# Autodesk Inventor assembly: Lift assembly left
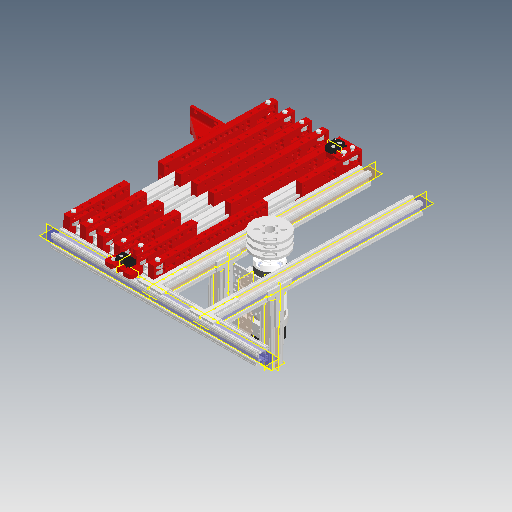
[picture p0: Inventor's stored thumbnail of the model, 512x512]
Saved by Autodesk Inventor 2020 (Build 240168000, 168)
## iProperties
Created: 2019-11-17
Part Number: Lift assembly left
Document SubType Name: Assembly
Designer: ball
Author: ball
## Documents named in this file (22)
- C:\FTC\FTC8863CAD\2019 Robot\Delivery\Lift assembly left.iam
- C:\FTC\FTC8863CAD\Actobotics\605 parts\605630.ipt
- C:\FTC\FTC8863CAD\StepLibraries\Nuts\2-56 NYLON-INSERT LOCKNUT.ipt
- C:\FTC\FTC8863CAD\StepLibraries\Screws\M3 x 25 HEX HEAD CAP SCREW.ipt
- C:\FTC\FTC8863CAD\2019 Robot\Delivery\Limit switch trigger spacer.ipt
- C:\FTC\FTC8863CAD\Actobotics\565 parts\565046.ipt
- C:\FTC\FTC8863CAD\Actobotics\585 parts\585075.ipt
- C:\FTC\FTC8863CAD\Actobotics\565 parts\xrail_3.5in.ipt
- C:\FTC\FTC8863CAD\Andymark\am-3461a NeveRest 4 with Motor REV3.ipt
- C:\FTC\FTC8863CAD\Actobotics\555 parts\555116 assembly.ipt
- C:\FTC\FTC8863CAD\2019 Robot\Generic Parts\limit switch mount to xrail.ipt
- C:\FTC\FTC8863CAD\StepLibraries\Screws\2-56x.5_18-8 SS PAN HEAD PHILLIPS MACHINE SCREW.ipt
- C:\FTC\FTC8863CAD\StepLibraries\Screws\6-32x.375_18-8 SS TRUSS HEAD PHILLIPS MACHINE SCREW.ipt
- C:\FTC\FTC8863CAD\2019 Robot\Delivery\Limit switch top + mount.iam
- C:\FTC\FTC8863CAD\2019 Robot\Delivery\Coupler lift long left bracket + pulleys.iam
- C:\FTC\FTC8863CAD\2019 Robot\Delivery\SAR330  x 5 + couplers left.iam
- C:\FTC\FTC8863CAD\2019 Robot\Delivery\Coupler lift short left + pulleys.iam
- C:\FTC\FTC8863CAD\Actobotics\615 parts\615468 inner plate.ipt
- C:\FTC\FTC8863CAD\Actobotics\615 parts\615468 outer plate 2_0 diameter.ipt
- C:\FTC\FTC8863CAD\Actobotics\545 parts\545619 assembly.ipt
- C:\FTC\FTC8863CAD\Actobotics\585 parts\585721.ipt
- C:\FTC\FTC8863CAD\2019 Robot\Delivery\Cross bar bracket.ipt
## Components (36 placed, 21 different names)
1. SAR330  x 5 + couplers left:1 [sub-assembly] — Mate:5, Flush:7, Mate:18, Mate:19, Mate:33, Mate:34, Mate:35, Mate:36, Flush:16, Mate:38, Flush:20, Mate:40, Flush:21, Flush:24, Mate:43, Flush:34, Flush:35, Mate:68, Mate:72, Mate:73, Mate:74
2. 605630:2 — Mate:5, Flush:7, Flush:33, Mate:61, Mate:63, Mate:64, Mate:65
3. M3 x 25 HEX HEAD CAP SCREW:1 — Mate:18, Mate:19, Mate:25, Mate:26
4. Limit switch trigger spacer:1 — Mate:25, Mate:26
5. M3 x 25 HEX HEAD CAP SCREW:2 — Mate:33
6. M3 x 25 HEX HEAD CAP SCREW:3 — Mate:34
7. Coupler lift short left + pulleys:1 [sub-assembly] — Mate:35, Mate:36, Flush:16, Flush:17, Flush:19, Mate:37
8. 565046:1 — Flush:17, Flush:19, Mate:37, Mate:39, Flush:22, Mate:42, Flush:25, Mate:48, Mate:49, Mate:60, Flush:32
9. 585075:1 — Mate:38, Flush:20, Mate:39
10. xrail_3.5in:1 — Mate:40, Flush:21, Flush:22, Mate:41, Flush:23, Flush:27, Symmetry:1, Flush:29
11. 585075:2 — Mate:41, Flush:23, Flush:24
12. 565046:2 — Mate:42, Flush:25, Mate:43, Mate:44, Flush:26, Mate:46, Flush:28, Mate:50, Mate:51, Mate:99
13. xrail_3.5in:2 — Mate:44, Flush:26, Flush:27, Mate:45, Mate:47, Mate:52, Symmetry:1, Mate:56, Mate:57, Mate:98, Mate:100, Mate:102
14. 585075:3 — Mate:45, Mate:46, Mate:47
15. 585075:4 — Mate:48, Flush:28, Mate:49
16. 585075:5 — Mate:50, Mate:51, Mate:52
17. am-3461a NeveRest 4 with Motor REV3:1 — Mate:53, Flush:29, Mate:54, Mate:55, Flush:30, Flush:31, Mate:90, Mate:91
18. 555116 assembly:1 — Mate:54, Flush:31
19. 555116 assembly:2 — Mate:55, Flush:30, Mate:56, Mate:57, Mate:103
20. limit switch mount to xrail:1 — Mate:60, Flush:32, Flush:33, Mate:61, Mate:62, Angle:1, Mate:66, Mate:67
21. 2-56 NYLON-INSERT LOCKNUT:4 — Mate:62, Mate:63, Angle:1
22. 2-56x.5_18-8 SS PAN HEAD PHILLIPS MACHINE SCREW:1 — Mate:64, Mate:65
23. 6-32x.375_18-8 SS TRUSS HEAD PHILLIPS MACHINE SCREW:1 — Mate:66, Mate:67
24. Limit switch top + mount:1 [sub-assembly] — Flush:34, Flush:35, Mate:68
25. Coupler lift long left bracket + pulleys:1 [sub-assembly] — Mate:72, Mate:73, Mate:74, Mate:104, Mate:105
26. 615468 inner plate:1 — Mate:76, Mate:77, Mate:78, Mate:79
27. 615468 outer plate 2_0 diameter:1 — Mate:78, Mate:79, Mate:84, Mate:85
28. 615468 inner plate:2 — Mate:76, Mate:77, Mate:80, Mate:81
29. 615468 outer plate 2_0 diameter:2 — Mate:80, Mate:81, Mate:91
30. 615468 inner plate:3 — Mate:82, Mate:83, Mate:84, Mate:86, Mate:87
31. 615468 inner plate:4 — Mate:82, Mate:83, Mate:85
32. 615468 outer plate 2_0 diameter:3 — Mate:86, Mate:87, Mate:88, Mate:89
33. 545619 assembly:1 — Mate:88, Mate:89, Mate:90
34. 585721:1 — Mate:98, Mate:99, Flush:38, Mate:101, Mate:103
35. 585721:2 — Mate:100, Flush:38, Mate:101, Mate:102
36. Cross bar bracke leftt:1 — Mate:104, Mate:105
## Relationships (89: Mate 66, Flush 21, Symmetry 1, Angle 1)
- Mate:5 (1.27 mm): SAR330  x 5 + couplers left:1 ↔ 605630:2
- Flush:7: SAR330  x 5 + couplers left:1 ↔ 605630:2
- Mate:18: SAR330  x 5 + couplers left:1 ↔ M3 x 25 HEX HEAD CAP SCREW:1
- Mate:19 (6 mm): SAR330  x 5 + couplers left:1 ↔ M3 x 25 HEX HEAD CAP SCREW:1
- Mate:25: M3 x 25 HEX HEAD CAP SCREW:1 ↔ Limit switch trigger spacer:1
- Mate:26: M3 x 25 HEX HEAD CAP SCREW:1 ↔ Limit switch trigger spacer:1
- Mate:33: SAR330  x 5 + couplers left:1 ↔ M3 x 25 HEX HEAD CAP SCREW:2
- Mate:34: SAR330  x 5 + couplers left:1 ↔ M3 x 25 HEX HEAD CAP SCREW:3
- Mate:35: SAR330  x 5 + couplers left:1 ↔ Coupler lift short left + pulleys:1
- Mate:36: SAR330  x 5 + couplers left:1 ↔ Coupler lift short left + pulleys:1
- Flush:16: SAR330  x 5 + couplers left:1 ↔ Coupler lift short left + pulleys:1
- Flush:17: Coupler lift short left + pulleys:1 ↔ 565046:1
- Flush:19: Coupler lift short left + pulleys:1 ↔ 565046:1
- Mate:37: Coupler lift short left + pulleys:1 ↔ 565046:1
- Mate:38: SAR330  x 5 + couplers left:1 ↔ 585075:1
- Flush:20: SAR330  x 5 + couplers left:1 ↔ 585075:1
- Mate:39: 565046:1 ↔ 585075:1
- Mate:40: SAR330  x 5 + couplers left:1 ↔ xrail_3.5in:1
- Flush:21: SAR330  x 5 + couplers left:1 ↔ xrail_3.5in:1
- Flush:22 (100.2792 mm): 565046:1 ↔ xrail_3.5in:1
- Mate:41: xrail_3.5in:1 ↔ 585075:2
- Flush:23: xrail_3.5in:1 ↔ 585075:2
- Flush:24: SAR330  x 5 + couplers left:1 ↔ 585075:2
- Mate:42: 565046:1 ↔ 565046:2
- Flush:25: 565046:1 ↔ 565046:2
- Mate:43 (57.15 mm): SAR330  x 5 + couplers left:1 ↔ 565046:2
- Mate:44: 565046:2 ↔ xrail_3.5in:2
- Flush:26: 565046:2 ↔ xrail_3.5in:2
- Flush:27: xrail_3.5in:1 ↔ xrail_3.5in:2
- Mate:45: xrail_3.5in:2 ↔ 585075:3
- Mate:46: 565046:2 ↔ 585075:3
- Mate:47: xrail_3.5in:2 ↔ 585075:3
- Mate:48: 565046:1 ↔ 585075:4
- Flush:28: 565046:2 ↔ 585075:4
- Mate:49: 565046:1 ↔ 585075:4
- Mate:50: 565046:2 ↔ 585075:5
- Mate:51: 565046:2 ↔ 585075:5
- Mate:52: xrail_3.5in:2 ↔ 585075:5
- Symmetry:1: xrail_3.5in:1 ↔ xrail_3.5in:2
- Mate:53: am-3461a NeveRest 4 with Motor REV3:1
- Flush:29: xrail_3.5in:1 ↔ am-3461a NeveRest 4 with Motor REV3:1
- Mate:54: am-3461a NeveRest 4 with Motor REV3:1 ↔ 555116 assembly:1
- Mate:55: am-3461a NeveRest 4 with Motor REV3:1 ↔ 555116 assembly:2
- Flush:30 (19.05 mm): am-3461a NeveRest 4 with Motor REV3:1 ↔ 555116 assembly:2
- Flush:31 (22.86 mm): am-3461a NeveRest 4 with Motor REV3:1 ↔ 555116 assembly:1
- Mate:56: xrail_3.5in:2 ↔ 555116 assembly:2
- Mate:57: xrail_3.5in:2 ↔ 555116 assembly:2
- Mate:60: 565046:1 ↔ limit switch mount to xrail:1
- Flush:32: 565046:1 ↔ limit switch mount to xrail:1
- Flush:33: 605630:2 ↔ limit switch mount to xrail:1
- Mate:61: 605630:2 ↔ limit switch mount to xrail:1
- Mate:62: limit switch mount to xrail:1 ↔ 2-56 NYLON-INSERT LOCKNUT:4
- Mate:63: 605630:2 ↔ 2-56 NYLON-INSERT LOCKNUT:4
- Angle:1 (0 deg): limit switch mount to xrail:1 ↔ 2-56 NYLON-INSERT LOCKNUT:4
- Mate:64: 605630:2 ↔ 2-56x.5_18-8 SS PAN HEAD PHILLIPS MACHINE SCREW:1
- Mate:65: 605630:2 ↔ 2-56x.5_18-8 SS PAN HEAD PHILLIPS MACHINE SCREW:1
- Mate:66: limit switch mount to xrail:1 ↔ 6-32x.375_18-8 SS TRUSS HEAD PHILLIPS MACHINE SCREW:1
- Mate:67: limit switch mount to xrail:1 ↔ 6-32x.375_18-8 SS TRUSS HEAD PHILLIPS MACHINE SCREW:1
- Flush:34: SAR330  x 5 + couplers left:1 ↔ Limit switch top + mount:1
- Flush:35 (2.54 mm): SAR330  x 5 + couplers left:1 ↔ Limit switch top + mount:1
- Mate:68: SAR330  x 5 + couplers left:1 ↔ Limit switch top + mount:1
- Mate:72: SAR330  x 5 + couplers left:1 ↔ Coupler lift long left bracket + pulleys:1
- Mate:73: SAR330  x 5 + couplers left:1 ↔ Coupler lift long left bracket + pulleys:1
- Mate:74: SAR330  x 5 + couplers left:1 ↔ Coupler lift long left bracket + pulleys:1
- Mate:76: 615468 inner plate:1 ↔ 615468 inner plate:2
- Mate:77: 615468 inner plate:1 ↔ 615468 inner plate:2
- Mate:78: 615468 inner plate:1 ↔ 615468 outer plate 2_0 diameter:1
- Mate:79: 615468 inner plate:1 ↔ 615468 outer plate 2_0 diameter:1
- Mate:80: 615468 inner plate:2 ↔ 615468 outer plate 2_0 diameter:2
- Mate:81: 615468 inner plate:2 ↔ 615468 outer plate 2_0 diameter:2
- Mate:82: 615468 inner plate:3 ↔ 615468 inner plate:4
- Mate:83: 615468 inner plate:3 ↔ 615468 inner plate:4
- Mate:84: 615468 outer plate 2_0 diameter:1 ↔ 615468 inner plate:3
- Mate:85: 615468 outer plate 2_0 diameter:1 ↔ 615468 inner plate:4
- Mate:86: 615468 inner plate:3 ↔ 615468 outer plate 2_0 diameter:3
- Mate:87: 615468 inner plate:3 ↔ 615468 outer plate 2_0 diameter:3
- Mate:88: 615468 outer plate 2_0 diameter:3 ↔ 545619 assembly:1
- Mate:89: 615468 outer plate 2_0 diameter:3 ↔ 545619 assembly:1
- Mate:90: am-3461a NeveRest 4 with Motor REV3:1 ↔ 545619 assembly:1
- Mate:91: am-3461a NeveRest 4 with Motor REV3:1 ↔ 615468 outer plate 2_0 diameter:2
- Mate:98: xrail_3.5in:2 ↔ 585721:1
- Mate:99: 565046:2 ↔ 585721:1
- Mate:100: xrail_3.5in:2 ↔ 585721:2
- Flush:38: 585721:1 ↔ 585721:2
- Mate:101: 585721:1 ↔ 585721:2
- Mate:102: xrail_3.5in:2 ↔ 585721:2
- Mate:103: 555116 assembly:2 ↔ 585721:1
- Mate:104: Coupler lift long left bracket + pulleys:1 ↔ Cross bar bracke leftt:1
- Mate:105: Coupler lift long left bracket + pulleys:1 ↔ Cross bar bracke leftt:1
